# Autodesk Inventor assembly: assembled-antenna
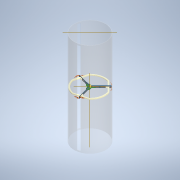
[picture p0: Inventor's stored thumbnail of the model, 180x180]
Saved by Autodesk Inventor 2021 (Build 250183000, 183)
## iProperties
Created: 2020-09-03
Part Number: assembled-antenna
Document SubType Name: Assembly
Designer: dsouthall
Author: dsouthall
## Documents named in this file (6)
- C:\Users\dsouthall\OneDrive - The University of Chicago\Hpol\hpol-prototype\design\Tri-Slot\Model 8 in\assembled-open-antenna.iam
- C:\Users\dsouthall\OneDrive - The University of Chicago\Hpol\hpol-prototype\design\Tri-Slot\Model 8 in\assembled-feed.iam
- C:\Users\dsouthall\OneDrive - The University of Chicago\Hpol\hpol-prototype\design\Tri-Slot\Model 8 in\source\92141A003_TYPE 18-8 STAINLESS STEEL FLAT WASHER\92141A003_TYPE 18-8 STAINLESS STEEL FLAT WASHER.ipt
- C:\Users\dsouthall\OneDrive - The University of Chicago\Hpol\hpol-prototype\design\Tri-Slot\Model 8 in\source\96877A118_18-8 SS 82 DEG FLAT HEAD PHIL MACHINE SCREW\96877A118_18-8 SS 82 DEG FLAT HEAD PHIL MACHINE SCREW.ipt
- C:\Users\dsouthall\OneDrive - The University of Chicago\Hpol\hpol-prototype\design\Tri-Slot\Model 8 in\source\91841A003_TYPE 18-8 STAINLESS STEEL HEX NUT\91841A003_TYPE 18-8 STAINLESS STEEL HEX NUT.ipt
- C:\Users\dsouthall\OneDrive - The University of Chicago\Hpol\hpol-prototype\design\Tri-Slot\Model 8 in\source\my can\can_open.ipt
## Components (20 placed, 5 different names)
1. can_open:1 — Insert:19, Insert:20, Insert:25, Insert:26, Insert:27, Insert:28, Mate:3, Mate:4, Mate:5
2. assembled-feed:1 [sub-assembly] — Mate:3, Mate:5
3. 96877A118_18-8 SS 82 DEG FLAT HEAD PHIL MACHINE SCREW:3 — Insert:26, Insert:35
4. 96877A118_18-8 SS 82 DEG FLAT HEAD PHIL MACHINE SCREW:4 — Insert:25, Insert:33
5. 96877A118_18-8 SS 82 DEG FLAT HEAD PHIL MACHINE SCREW:5 — Insert:28, Insert:29
6. 96877A118_18-8 SS 82 DEG FLAT HEAD PHIL MACHINE SCREW:6 — Insert:27, Insert:30
7. 92141A003_TYPE 18-8 STAINLESS STEEL FLAT WASHER:9 — Insert:30, Insert:32
8. 92141A003_TYPE 18-8 STAINLESS STEEL FLAT WASHER:10 — Insert:29, Insert:31
9. 92141A003_TYPE 18-8 STAINLESS STEEL FLAT WASHER:11 — Insert:33, Insert:34
10. 92141A003_TYPE 18-8 STAINLESS STEEL FLAT WASHER:12 — Insert:35, Insert:36
11. 91841A003_TYPE 18-8 STAINLESS STEEL HEX NUT:3 — Insert:36
12. 91841A003_TYPE 18-8 STAINLESS STEEL HEX NUT:4 — Insert:34
13. 91841A003_TYPE 18-8 STAINLESS STEEL HEX NUT:5 — Insert:31
14. 91841A003_TYPE 18-8 STAINLESS STEEL HEX NUT:6 — Insert:32
15. 96877A118_18-8 SS 82 DEG FLAT HEAD PHIL MACHINE SCREW:1 — Insert:19, Insert:21
16. 96877A118_18-8 SS 82 DEG FLAT HEAD PHIL MACHINE SCREW:2 — Insert:20, Insert:23
17. 92141A003_TYPE 18-8 STAINLESS STEEL FLAT WASHER:7 — Insert:23, Insert:24
18. 92141A003_TYPE 18-8 STAINLESS STEEL FLAT WASHER:8 — Insert:21, Insert:22
19. 91841A003_TYPE 18-8 STAINLESS STEEL HEX NUT:1 — Insert:24
20. 91841A003_TYPE 18-8 STAINLESS STEEL HEX NUT:2 — Insert:22
## Relationships (21: Insert 18, Mate 3)
- Insert:19: can_open:1 ↔ 96877A118_18-8 SS 82 DEG FLAT HEAD PHIL MACHINE SCREW:1
- Insert:20: can_open:1 ↔ 96877A118_18-8 SS 82 DEG FLAT HEAD PHIL MACHINE SCREW:2
- Insert:21 (-2.54 mm): 96877A118_18-8 SS 82 DEG FLAT HEAD PHIL MACHINE SCREW:1 ↔ 92141A003_TYPE 18-8 STAINLESS STEEL FLAT WASHER:8
- Insert:22: 92141A003_TYPE 18-8 STAINLESS STEEL FLAT WASHER:8 ↔ 91841A003_TYPE 18-8 STAINLESS STEEL HEX NUT:2
- Insert:23 (-2.54 mm): 96877A118_18-8 SS 82 DEG FLAT HEAD PHIL MACHINE SCREW:2 ↔ 92141A003_TYPE 18-8 STAINLESS STEEL FLAT WASHER:7
- Insert:24: 92141A003_TYPE 18-8 STAINLESS STEEL FLAT WASHER:7 ↔ 91841A003_TYPE 18-8 STAINLESS STEEL HEX NUT:1
- Insert:25: can_open:1 ↔ 96877A118_18-8 SS 82 DEG FLAT HEAD PHIL MACHINE SCREW:4
- Insert:26: can_open:1 ↔ 96877A118_18-8 SS 82 DEG FLAT HEAD PHIL MACHINE SCREW:3
- Insert:27: can_open:1 ↔ 96877A118_18-8 SS 82 DEG FLAT HEAD PHIL MACHINE SCREW:6
- Insert:28: can_open:1 ↔ 96877A118_18-8 SS 82 DEG FLAT HEAD PHIL MACHINE SCREW:5
- Insert:29 (-2.54 mm): 96877A118_18-8 SS 82 DEG FLAT HEAD PHIL MACHINE SCREW:5 ↔ 92141A003_TYPE 18-8 STAINLESS STEEL FLAT WASHER:10
- Insert:30 (-2.54 mm): 96877A118_18-8 SS 82 DEG FLAT HEAD PHIL MACHINE SCREW:6 ↔ 92141A003_TYPE 18-8 STAINLESS STEEL FLAT WASHER:9
- Insert:31: 92141A003_TYPE 18-8 STAINLESS STEEL FLAT WASHER:10 ↔ 91841A003_TYPE 18-8 STAINLESS STEEL HEX NUT:5
- Insert:32: 92141A003_TYPE 18-8 STAINLESS STEEL FLAT WASHER:9 ↔ 91841A003_TYPE 18-8 STAINLESS STEEL HEX NUT:6
- Insert:33 (-2.54 mm): 96877A118_18-8 SS 82 DEG FLAT HEAD PHIL MACHINE SCREW:4 ↔ 92141A003_TYPE 18-8 STAINLESS STEEL FLAT WASHER:11
- Insert:34: 92141A003_TYPE 18-8 STAINLESS STEEL FLAT WASHER:11 ↔ 91841A003_TYPE 18-8 STAINLESS STEEL HEX NUT:4
- Insert:35 (-2.54 mm): 96877A118_18-8 SS 82 DEG FLAT HEAD PHIL MACHINE SCREW:3 ↔ 92141A003_TYPE 18-8 STAINLESS STEEL FLAT WASHER:12
- Insert:36: 92141A003_TYPE 18-8 STAINLESS STEEL FLAT WASHER:12 ↔ 91841A003_TYPE 18-8 STAINLESS STEEL HEX NUT:3
- Mate:3: can_open:1 ↔ assembled-feed:1
- Mate:4 (600 mm): can_open:1
- Mate:5 (300 mm): can_open:1 ↔ assembled-feed:1
